# Autodesk Inventor assembly: Panel B
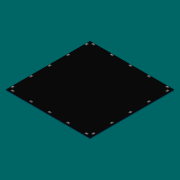
[picture p0: Inventor's stored thumbnail of the model, 180x180]
Saved by Autodesk Inventor 2016 (Build 200138000, 138)
## iProperties
Created: 2015-06-04
Part Number: Panel B
Document SubType Name: Assembly
Designer: Sawaiz Syed
Author: Sawaiz Syed
## Documents named in this file (4)
- C:\Users\Sawaiz\Documents\data\projects\cncBlackBox\panels\panelB.iam
- C:\Users\Sawaiz\Documents\data\projects\cncBlackBox\panels\faceBFelt.ipt
- C:\Users\Sawaiz\Documents\data\projects\cncBlackBox\panels\faceB.ipt
- C:\Users\Sawaiz\Documents\data\projects\cncBlackBox\panels\facingScrew.iam
## Components (22 placed, 3 different names)
1. faceB:1 — Mate:1, Mate:2, Flush:1, Mate:3, Mate:4, Angle:1, Mate:5, Angle:2, Mate:6
2. faceBFelt:1 — Mate:1, Mate:2, Flush:1
3. facingScrew:1 [sub-assembly] — Mate:3
4. facingScrew:2 [sub-assembly]
5. facingScrew:3 [sub-assembly]
6. facingScrew:4 [sub-assembly] — Mate:4
7. facingScrew:5 [sub-assembly]
8. facingScrew:7 [sub-assembly]
9. facingScrew:8 [sub-assembly]
10. facingScrew:9 [sub-assembly]
11. facingScrew:10 [sub-assembly] — Angle:1
12. facingScrew:11 [sub-assembly]
13. facingScrew:6 [sub-assembly] — Mate:5, Angle:2, Mate:6
14. facingScrew:12 [sub-assembly]
15. facingScrew:13 [sub-assembly]
16. facingScrew:14 [sub-assembly]
17. facingScrew:15 [sub-assembly]
18. facingScrew:16 [sub-assembly]
19. facingScrew:17 [sub-assembly]
20. facingScrew:18 [sub-assembly]
21. facingScrew:19 [sub-assembly]
22. facingScrew:20 [sub-assembly]
## Component patterns: (10 elements, first: facingScrew:1), (10 elements, first: facingScrew:6)
## Relationships (9: Mate 6, Angle 2, Flush 1)
- Mate:1: faceB:1 ↔ faceBFelt:1
- Mate:2: faceB:1 ↔ faceBFelt:1
- Flush:1: faceB:1 ↔ faceBFelt:1
- Mate:3: faceB:1 ↔ facingScrew:1
- Mate:4: faceB:1 ↔ facingScrew:4
- Angle:1 (0 deg): faceB:1 ↔ facingScrew:10
- Mate:5: faceB:1 ↔ facingScrew:6
- Angle:2 (0 deg): faceB:1 ↔ facingScrew:6
- Mate:6: faceB:1 ↔ facingScrew:6
